# Autodesk Inventor assembly: Updated Servo Arm
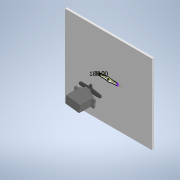
[picture p0: Inventor's stored thumbnail of the model, 180x180]
Saved by Autodesk Inventor 2020 (Build 240168000, 168)
## iProperties
Created: 2020-03-17
Part Number: Updated Servo Arm
Document SubType Name: Assembly
Designer: varun
Author: varun
## iProperties of the stored document MG90servo_shaft.ipt
Created: 2016-03-21
Part Number: MG90servo_shaft
Material: Generic
Document SubType Name: Modeling
Designer: varun
Density: 1 g/cm^3
Appearance: Default
Author: varun
Sending System: SolidWorks 2015
Last Author: Vitto
Last Saved: 2016-03-21
## iProperties of the stored document MG90servo_gear.ipt
Created: 2016-03-21
Part Number: MG90servo_gear
Material: Generic
Document SubType Name: Modeling
Designer: varun
Density: 1 g/cm^3
Appearance: Default
Author: varun
Sending System: SolidWorks 2015
Last Author: Vitto
Last Saved: 2016-03-21
## iProperties of the stored document MG90servo_assembly.iam
Created: 2016-03-21
Part Number: MG90servo_assembly
Document SubType Name: Assembly
Designer: varun
Author: varun
Sending System: SolidWorks 2015
Last Author: Vitto
Last Saved: 2016-03-21
## iProperties of the stored document MG90servo_body.ipt
Created: 2016-03-21
Part Number: MG90servo_body
Material: Generic
Document SubType Name: Modeling
Designer: varun
Density: 1 g/cm^3
Appearance: Default
Author: varun
Sending System: SolidWorks 2015
Last Author: Vitto
Last Saved: 2016-03-21
## Documents named in this file (10)
- **C:\Users\varun\Desktop\ServoArm\Updated Servo Arm.iam*LocalDocs*xAaaaaldaAaaaaaaaAaaaqrggQd*MG90servo_shaft.ipt
- **C:\Users\varun\Desktop\ServoArm\Updated Servo Arm.iam*LocalDocs*xAaaaaidaAaaaaaaaAaaaaljaPh*MG90servo_gear.ipt
- **C:\Users\varun\Desktop\ServoArm\Updated Servo Arm.iam*LocalDocs*xAaaaaedaAaaaaaaaAaaaqgv54g*MG90servo_assembly.iam
- **C:\Users\varun\Desktop\ServoArm\Updated Servo Arm.iam*LocalDocs*xAaaaqkbaAaaaaaaaAaaaqgphIf*MG90servo_body.ipt
- C:\Users\varun\Desktop\ServoArm\Updated Servo Arm.iam
- C:\Users\varun\Desktop\ServoArm\Base.ipt
- C:\Users\varun\Desktop\ServoArm\MG90servo_assembly.SLDASM
- C:\Users\varun\Desktop\ServoArm\MG90servo_body.SLDPRT
- C:\Users\varun\Desktop\ServoArm\MG90servo_gear.SLDPRT
- C:\Users\varun\Desktop\ServoArm\MG90servo_shaft.SLDPRT
## Components (2 placed, 2 different names)
1. Base:1 — Mate:1
2. MG90servo_assembly:1 [sub-assembly] — Mate:1
## Relationships (1: Mate 1)
- Mate:1: Base:1 ↔ MG90servo_assembly:1
